# Autodesk Inventor assembly: Fixed
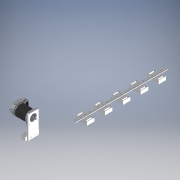
[picture p0: Inventor's stored thumbnail of the model, 180x180]
Saved by Autodesk Inventor 2016 (Build 200138000, 138)
## iProperties
Created: 2015-06-08
Part Number: Fixed
Document SubType Name: Assembly
Designer: Dennis
Author: Dennis
## Documents named in this file (6)
- C:\Users\Dennis\Dropbox\NI Work\NI Slider Crank\Assemblies\Fixed Parts.iam
- C:\Users\Dennis\Dropbox\NI Work\NI Slider Crank\Parts\Track Foot.ipt
- C:\Users\Dennis\Dropbox\NI Work\NI Slider Crank\Parts\Carriage Rail - 9829K134.ipt
- C:\Users\Dennis\Dropbox\NI Work\NI Slider Crank\Parts\Motor Support.ipt
- C:\Users\Dennis\Dropbox\NI Work\NI Slider Crank\Parts\Motor Base.ipt
- C:\Users\Dennis\Dropbox\NI Work\NI Slider Crank\Parts\Motor - CPM-_ _ _ _ - 2321_-Q_.ipt
## Components (9 placed, 5 different names)
1. Track Foot:1 — Mate:11, Mate:12
2. Track Foot:2 — Mate:13, Mate:26
3. Track Foot:3 — Mate:14, Mate:28
4. Track Foot:4 — Mate:15, Mate:29
5. Track Foot:5 — Mate:16, Mate:30
6. Carriage Rail - 9829K134:1 — Mate:11, Mate:12, Mate:13, Mate:14, Mate:15, Mate:16, Mate:18, Mate:19, Mate:26, Mate:28, Mate:29, Mate:30
7. Motor Support:1 — Mate:18, Mate:19, Mate:21, Mate:22, Mate:23, Mate:24, Angle:1
8. Motor Base:1 — Mate:21, Mate:22
9. Motor - CPM-_ _ _ _ - 2321_-Q_:1 — Mate:23, Mate:24, Angle:1
## Relationships (17: Mate 16, Angle 1)
- Mate:11: Track Foot:1 ↔ Carriage Rail - 9829K134:1
- Mate:12: Track Foot:1 ↔ Carriage Rail - 9829K134:1
- Mate:13: Track Foot:2 ↔ Carriage Rail - 9829K134:1
- Mate:14: Track Foot:3 ↔ Carriage Rail - 9829K134:1
- Mate:15: Track Foot:4 ↔ Carriage Rail - 9829K134:1
- Mate:16: Track Foot:5 ↔ Carriage Rail - 9829K134:1
- Mate:18 (53.5178 mm): Carriage Rail - 9829K134:1 ↔ Motor Support:1
- Mate:19 (139.7 mm): Carriage Rail - 9829K134:1 ↔ Motor Support:1
- Mate:21: Motor Support:1 ↔ Motor Base:1
- Mate:22: Motor Support:1 ↔ Motor Base:1
- Mate:23: Motor Support:1 ↔ Motor - CPM-_ _ _ _ - 2321_-Q_:1
- Mate:24: Motor Support:1 ↔ Motor - CPM-_ _ _ _ - 2321_-Q_:1
- Angle:1 (270 deg): Motor Support:1 ↔ Motor - CPM-_ _ _ _ - 2321_-Q_:1
- Mate:26: Track Foot:2 ↔ Carriage Rail - 9829K134:1
- Mate:28: Track Foot:3 ↔ Carriage Rail - 9829K134:1
- Mate:29: Track Foot:4 ↔ Carriage Rail - 9829K134:1
- Mate:30: Track Foot:5 ↔ Carriage Rail - 9829K134:1
